# Autodesk Inventor assembly: BG203_trajan20_21
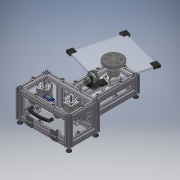
[picture p0: Inventor's stored thumbnail of the model, 180x180]
Saved by Autodesk Inventor 2022.2 (Build 262287000, 287)
## iProperties
Company: HTBLA Kaindorf
RuleStatus: InUse
Created: 2022-09-09
Part Number: BG203_trajan20_21
Project: Zeichenmaschine_v2
Material: Generisch
Description: Gerüst mit Papierplatte und Seitenwänden
Document SubType Name: Assembly
Designer: trajan20
AfterDocNew0: iProperties-Editor_aufrufen
Author: jan
Keywords: 2021
## Documents named in this file (9)
- C:\Users\jan\Documents\DrawMachine\DrawMachineConstruction\Projekt\Zeichenmaschine_v2\BG203_trajan20_21_Zeichenmaschine_v2_Gerüst mit Papierplatte und Seitenwänden.iam
- C:\Users\jan\Documents\DrawMachine\DrawMachineConstruction\Projekt\Zeichenmaschine_v2\BG202_trajan20_21_Zeichenmaschine_v2_Gerüst mit Motoren und Laufrolle.iam
- C:\Users\jan\Documents\DrawMachine\DrawMachineConstruction\Projekt\Zeichenmaschine_v2\BG401_trajan20_21_Zeichenmaschine_v2_papierplatte.iam
- C:\Users\jan\Documents\DrawMachine\DrawMachineConstruction\Projekt\Zeichenmaschine_v2\Normteile\de-DE\ISO 4029\ISO 4029 - M5 x 16 - ISO.ipt
- C:\Users\jan\Documents\DrawMachine\DrawMachineConstruction\Projekt\Zeichenmaschine_v2\BT701_trajan20_21_Zeichenmaschine_v2_Plexi_100x80.ipt
- C:\Users\jan\Documents\DrawMachine\DrawMachineConstruction\Projekt\Zeichenmaschine_v2\BT706_trajan20_21_Zeichenmaschine_v2_Plexi_100x80_nothalt.ipt
- C:\Users\jan\Documents\DrawMachine\DrawMachineConstruction\Projekt\Zeichenmaschine_v2\BT702_trajan20_21_Zeichenmaschine_v2_Plexi_40x80.ipt
- C:\Users\jan\Documents\DrawMachine\DrawMachineConstruction\Projekt\Zeichenmaschine_v2\BT704_trajan20_21_Zeichenmaschine_v2_Plexi_220x30.ipt
- C:\Users\jan\Documents\DrawMachine\DrawMachineConstruction\Projekt\Zeichenmaschine_v2\BT705_trajan20_21_Zeichenmaschine_v2_Plexi_80x30.ipt
## Components (10 placed, 8 different names)
1. BG202_trajan20_21_Zeichenmaschine_v2_Gerüst mit Motoren und Laufrolle:1 [sub-assembly] — Passend:1, Passend:2, Passend:8, Passend:9, Passend:10, Passend:11, Passend:12, Passend:13, Passend:14, Passend:15, Passend:16, Passend:17, Passend:18, Passend:19, Passend:20, Passend:21, Passend:22, Passend:23, Passend:24, Passend:25, Passend:26, Passend:27, Passend:28
2. BG401_trajan20_21_Zeichenmaschine_v2_papierplatte:1 [sub-assembly] — Passend:1, Passend:2, Passend:3, Passend:4
3. ISO 4029 M5 x 16:1 — Passend:3, Passend:4
4. BT701_trajan20_21_Zeichenmaschine_v2_Plexi_100x80:2 — Passend:8, Passend:9, Passend:10
5. BT706_trajan20_21_Zeichenmaschine_v2_Plexi_100x80_nothalt:1 — Passend:11, Passend:12, Passend:13
6. BT702_trajan20_21_Zeichenmaschine_v2_Plexi_40x80:1 — Passend:14, Passend:15, Passend:16
7. BT702_trajan20_21_Zeichenmaschine_v2_Plexi_40x80:2 — Passend:17, Passend:18, Passend:19
8. BT704_trajan20_21_Zeichenmaschine_v2_Plexi_220x30:1 — Passend:20, Passend:21, Passend:22
9. BT704_trajan20_21_Zeichenmaschine_v2_Plexi_220x30:2 — Passend:23, Passend:24, Passend:25
10. BT705_trajan20_21_Zeichenmaschine_v2_Plexi_80x30:1 — Passend:26, Passend:27, Passend:28
## Relationships (25: Mate 25)
- Passend:1 [Mate]: BG202_trajan20_21_Zeichenmaschine_v2_Gerüst mit Motoren und Laufrolle:1 ↔ BG401_trajan20_21_Zeichenmaschine_v2_papierplatte:1
- Passend:2 [Mate] (0.5 mm): BG202_trajan20_21_Zeichenmaschine_v2_Gerüst mit Motoren und Laufrolle:1 ↔ BG401_trajan20_21_Zeichenmaschine_v2_papierplatte:1
- Passend:3 [Mate]: BG401_trajan20_21_Zeichenmaschine_v2_papierplatte:1 ↔ ISO 4029 M5 x 16:1
- Passend:4 [Mate] (-17.5 mm): BG401_trajan20_21_Zeichenmaschine_v2_papierplatte:1 ↔ ISO 4029 M5 x 16:1
- Passend:8 [Mate]: BG202_trajan20_21_Zeichenmaschine_v2_Gerüst mit Motoren und Laufrolle:1 ↔ BT701_trajan20_21_Zeichenmaschine_v2_Plexi_100x80:2
- Passend:9 [Mate] (0.5 mm): BG202_trajan20_21_Zeichenmaschine_v2_Gerüst mit Motoren und Laufrolle:1 ↔ BT701_trajan20_21_Zeichenmaschine_v2_Plexi_100x80:2
- Passend:10 [Mate] (0.5 mm): BG202_trajan20_21_Zeichenmaschine_v2_Gerüst mit Motoren und Laufrolle:1 ↔ BT701_trajan20_21_Zeichenmaschine_v2_Plexi_100x80:2
- Passend:11 [Mate]: BG202_trajan20_21_Zeichenmaschine_v2_Gerüst mit Motoren und Laufrolle:1 ↔ BT706_trajan20_21_Zeichenmaschine_v2_Plexi_100x80_nothalt:1
- Passend:12 [Mate] (0.5 mm): BG202_trajan20_21_Zeichenmaschine_v2_Gerüst mit Motoren und Laufrolle:1 ↔ BT706_trajan20_21_Zeichenmaschine_v2_Plexi_100x80_nothalt:1
- Passend:13 [Mate] (0.5 mm): BG202_trajan20_21_Zeichenmaschine_v2_Gerüst mit Motoren und Laufrolle:1 ↔ BT706_trajan20_21_Zeichenmaschine_v2_Plexi_100x80_nothalt:1
- Passend:14 [Mate]: BG202_trajan20_21_Zeichenmaschine_v2_Gerüst mit Motoren und Laufrolle:1 ↔ BT702_trajan20_21_Zeichenmaschine_v2_Plexi_40x80:1
- Passend:15 [Mate] (0.5 mm): BG202_trajan20_21_Zeichenmaschine_v2_Gerüst mit Motoren und Laufrolle:1 ↔ BT702_trajan20_21_Zeichenmaschine_v2_Plexi_40x80:1
- Passend:16 [Mate] (0.5 mm): BG202_trajan20_21_Zeichenmaschine_v2_Gerüst mit Motoren und Laufrolle:1 ↔ BT702_trajan20_21_Zeichenmaschine_v2_Plexi_40x80:1
- Passend:17 [Mate] (0.5 mm): BG202_trajan20_21_Zeichenmaschine_v2_Gerüst mit Motoren und Laufrolle:1 ↔ BT702_trajan20_21_Zeichenmaschine_v2_Plexi_40x80:2
- Passend:18 [Mate]: BG202_trajan20_21_Zeichenmaschine_v2_Gerüst mit Motoren und Laufrolle:1 ↔ BT702_trajan20_21_Zeichenmaschine_v2_Plexi_40x80:2
- Passend:19 [Mate] (0.5 mm): BG202_trajan20_21_Zeichenmaschine_v2_Gerüst mit Motoren und Laufrolle:1 ↔ BT702_trajan20_21_Zeichenmaschine_v2_Plexi_40x80:2
- Passend:20 [Mate] (0.5 mm): BG202_trajan20_21_Zeichenmaschine_v2_Gerüst mit Motoren und Laufrolle:1 ↔ BT704_trajan20_21_Zeichenmaschine_v2_Plexi_220x30:1
- Passend:21 [Mate]: BG202_trajan20_21_Zeichenmaschine_v2_Gerüst mit Motoren und Laufrolle:1 ↔ BT704_trajan20_21_Zeichenmaschine_v2_Plexi_220x30:1
- Passend:22 [Mate] (0.5 mm): BG202_trajan20_21_Zeichenmaschine_v2_Gerüst mit Motoren und Laufrolle:1 ↔ BT704_trajan20_21_Zeichenmaschine_v2_Plexi_220x30:1
- Passend:23 [Mate]: BG202_trajan20_21_Zeichenmaschine_v2_Gerüst mit Motoren und Laufrolle:1 ↔ BT704_trajan20_21_Zeichenmaschine_v2_Plexi_220x30:2
- Passend:24 [Mate] (0.5 mm): BG202_trajan20_21_Zeichenmaschine_v2_Gerüst mit Motoren und Laufrolle:1 ↔ BT704_trajan20_21_Zeichenmaschine_v2_Plexi_220x30:2
- Passend:25 [Mate] (0.5 mm): BG202_trajan20_21_Zeichenmaschine_v2_Gerüst mit Motoren und Laufrolle:1 ↔ BT704_trajan20_21_Zeichenmaschine_v2_Plexi_220x30:2
- Passend:26 [Mate]: BG202_trajan20_21_Zeichenmaschine_v2_Gerüst mit Motoren und Laufrolle:1 ↔ BT705_trajan20_21_Zeichenmaschine_v2_Plexi_80x30:1
- Passend:27 [Mate] (0.5 mm): BG202_trajan20_21_Zeichenmaschine_v2_Gerüst mit Motoren und Laufrolle:1 ↔ BT705_trajan20_21_Zeichenmaschine_v2_Plexi_80x30:1
- Passend:28 [Mate] (0.5 mm): BG202_trajan20_21_Zeichenmaschine_v2_Gerüst mit Motoren und Laufrolle:1 ↔ BT705_trajan20_21_Zeichenmaschine_v2_Plexi_80x30:1
